# Autodesk Inventor assembly: Progres IoT 3iam
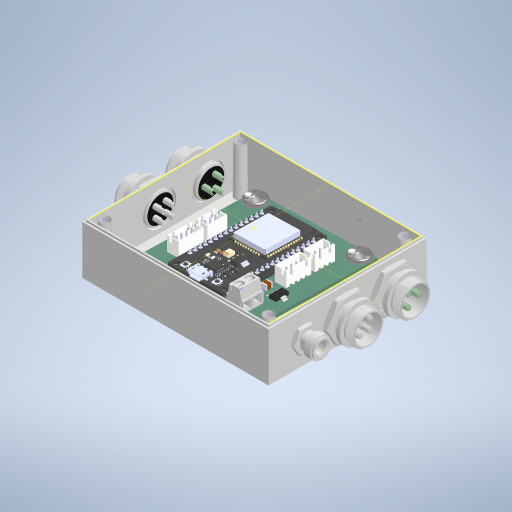
[picture p0: Inventor's stored thumbnail of the model, 512x512]
Saved by Autodesk Inventor 2023 (Build 270158000, 158)
## iProperties
Company: Kicad
Created: 2024-10-20
Part Number: Progres IoT 3iam
Description: KiCad electronic assembly
Document SubType Name: Assembly
Designer: Juan
Authority: Unknown
Sending System: KiCad to STEP converter
Preprocessor: Open CASCADE STEP processor 7.8
Title: aquasmart.step
Author: Pcbnew
## Documents named in this file (7)
- D:\Semester 5\IoT dan Jaringan Sensor\aquasmart\aquasmart\progres 3\Progres IoT 3iam.iam
- D:\Semester 5\IoT dan Jaringan Sensor\aquasmart\aquasmart\progres 2\ProjectIOT2.ipt
- C:\Users\Juan\Downloads\gx-16-connector-4-pins-1.snapshot.3 (1)\GX-16 Connector 4 Pins.iam
- C:\Users\Juan\Downloads\gx-16-connector-3-pins-1.snapshot.3\GX-16 Connector 3 Pins.iam
- C:\Users\Juan\Downloads\dc-power-jack-2-1mm-socket-female-panel-mount-1.snapshot.2\DJ Jack 2,1mm panel mount.ipt
- C:\Users\Juan\Downloads\revisi.iam
- C:\Users\Juan\Documents\Inventor\Content Center Files\R2023\en-US\AS 1427(05)\AS 1427 - M5 x 6(5) II.ipt
## Components (11 placed, 6 different names)
1. ProjectIOT2:1 — Insert:2, Insert:3, Insert:6, Mate:2, Insert:11, Insert:12
2. GX-16 Connector 4 Pins:1 [sub-assembly] — Insert:2
3. GX-16 Connector 4 Pins:2 [sub-assembly] — Insert:3
4. DJ Jack 2,1mm panel mount:1 — Insert:6
5. revisi:1 [sub-assembly] — Mate:2, Insert:7, Insert:8, Insert:9, Insert:10
6. AS 1427 H - Metric M5 x 6:1 — Insert:7
7. AS 1427 H - Metric M5 x 6:2 — Insert:8
8. AS 1427 H - Metric M5 x 6:3 — Insert:9
9. AS 1427 H - Metric M5 x 6:4 — Insert:10
10. GX-16 Connector 3 Pins:1 [sub-assembly] — Insert:11
11. GX-16 Connector 3 Pins:2 [sub-assembly] — Insert:12
## Relationships (10: Insert 9, Mate 1)
- Insert:2: ProjectIOT2:1 ↔ GX-16 Connector 4 Pins:1
- Insert:3 (-2 mm): ProjectIOT2:1 ↔ GX-16 Connector 4 Pins:2
- Insert:6: ProjectIOT2:1 ↔ DJ Jack 2,1mm panel mount:1
- Mate:2: ProjectIOT2:1 ↔ revisi:1
- Insert:7: revisi:1 ↔ AS 1427 H - Metric M5 x 6:1
- Insert:8: revisi:1 ↔ AS 1427 H - Metric M5 x 6:2
- Insert:9: revisi:1 ↔ AS 1427 H - Metric M5 x 6:3
- Insert:10: revisi:1 ↔ AS 1427 H - Metric M5 x 6:4
- Insert:11: ProjectIOT2:1 ↔ GX-16 Connector 3 Pins:1
- Insert:12: ProjectIOT2:1 ↔ GX-16 Connector 3 Pins:2
